# Autodesk Inventor assembly: assembly
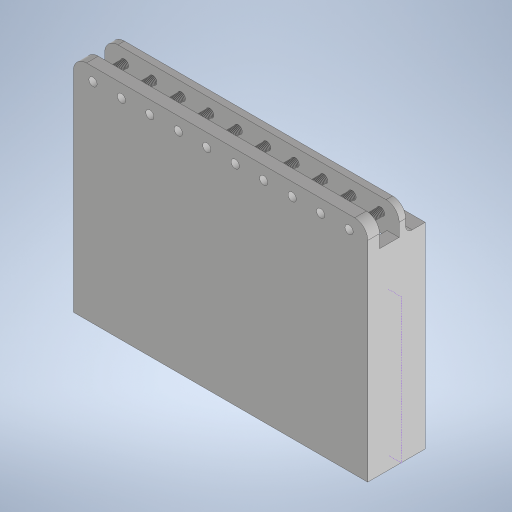
[picture p0: Inventor's stored thumbnail of the model, 512x512]
Saved by Autodesk Inventor 2024.3 (Build 283343000, 343)
## iProperties
Created: 2025-01-01
Part Number: assembly
Document SubType Name: Assembly
Designer: email
Author: email
## Documents named in this file (6)
- C:\Users\email\Desktop\Projects\Capstone\electornicsbox\assembly.iam
- C:\Users\email\Desktop\Projects\Capstone\electornicsbox\ebox.ipt
- C:\Users\email\Desktop\Projects\Capstone\electornicsbox\arduinomega.ipt
- C:\Users\email\Desktop\Projects\Capstone\electornicsbox\hx711.ipt
- C:\Users\email\Desktop\Projects\Capstone\electornicsbox\motorcontroller.ipt
- C:\Users\email\Documents\Inventor\Content Center Files\R2021\en-US\ISO 7380-1\ISO 7380-1 - M6 x 25.ipt
## Components (14 placed, 5 different names)
1. ebox:1 — Mate:1, Mate:2, Mate:3, Mate:4, Mate:5, Mate:6, Mate:11, Mate:12, Mate:13, Mate:14, Mate:15, Mate:16, Mate:17, Mate:18, Mate:19, Mate:20, Mate:21, Mate:22, Mate:23, Mate:24, Mate:25, Mate:26, Mate:27, Mate:28, Mate:29, Mate:30, Mate:31, Mate:32, Mate:33, Mate:34, Mate:35, Mate:36, Mate:37
2. arduinomega:1 — Mate:1, Mate:2, Mate:3, Mate:4, Mate:5
3. hx711:1 — Mate:11, Mate:12, Mate:13
4. motorcontroller:1 — Mate:6, Mate:34, Mate:35, Mate:36, Mate:37
5. ISO 7380-1 M6 x 25:1 — Mate:16, Mate:17
6. ISO 7380-1 M6 x 25:2 — Mate:14, Mate:15
7. ISO 7380-1 M6 x 25:3 — Mate:18, Mate:19
8. ISO 7380-1 M6 x 25:4 — Mate:20, Mate:21
9. ISO 7380-1 M6 x 25:5 — Mate:22, Mate:23
10. ISO 7380-1 M6 x 25:6 — Mate:24, Mate:25
11. ISO 7380-1 M6 x 25:7 — Mate:26, Mate:27
12. ISO 7380-1 M6 x 25:8 — Mate:28, Mate:29
13. ISO 7380-1 M6 x 25:9 — Mate:30, Mate:31
14. ISO 7380-1 M6 x 25:10 — Mate:32, Mate:33
## Relationships (33: Mate 33)
- Mate:1: ebox:1 ↔ arduinomega:1
- Mate:2: ebox:1 ↔ arduinomega:1
- Mate:3: ebox:1 ↔ arduinomega:1
- Mate:4: ebox:1 ↔ arduinomega:1
- Mate:5: ebox:1 ↔ arduinomega:1
- Mate:6: ebox:1 ↔ motorcontroller:1
- Mate:11: ebox:1 ↔ hx711:1
- Mate:12: ebox:1 ↔ hx711:1
- Mate:13: ebox:1 ↔ hx711:1
- Mate:14: ebox:1 ↔ ISO 7380-1 M6 x 25:2
- Mate:15: ebox:1 ↔ ISO 7380-1 M6 x 25:2
- Mate:16: ebox:1 ↔ ISO 7380-1 M6 x 25:1
- Mate:17: ebox:1 ↔ ISO 7380-1 M6 x 25:1
- Mate:18: ebox:1 ↔ ISO 7380-1 M6 x 25:3
- Mate:19: ebox:1 ↔ ISO 7380-1 M6 x 25:3
- Mate:20: ebox:1 ↔ ISO 7380-1 M6 x 25:4
- Mate:21: ebox:1 ↔ ISO 7380-1 M6 x 25:4
- Mate:22: ebox:1 ↔ ISO 7380-1 M6 x 25:5
- Mate:23: ebox:1 ↔ ISO 7380-1 M6 x 25:5
- Mate:24: ebox:1 ↔ ISO 7380-1 M6 x 25:6
- Mate:25: ebox:1 ↔ ISO 7380-1 M6 x 25:6
- Mate:26: ebox:1 ↔ ISO 7380-1 M6 x 25:7
- Mate:27: ebox:1 ↔ ISO 7380-1 M6 x 25:7
- Mate:28: ebox:1 ↔ ISO 7380-1 M6 x 25:8
- Mate:29: ebox:1 ↔ ISO 7380-1 M6 x 25:8
- Mate:30: ebox:1 ↔ ISO 7380-1 M6 x 25:9
- Mate:31: ebox:1 ↔ ISO 7380-1 M6 x 25:9
- Mate:32: ebox:1 ↔ ISO 7380-1 M6 x 25:10
- Mate:33: ebox:1 ↔ ISO 7380-1 M6 x 25:10
- Mate:34: ebox:1 ↔ motorcontroller:1
- Mate:35: ebox:1 ↔ motorcontroller:1
- Mate:36: ebox:1 ↔ motorcontroller:1
- Mate:37: ebox:1 ↔ motorcontroller:1
